# Autodesk Inventor assembly: Lower_wheel
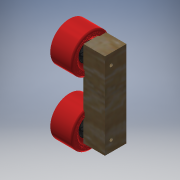
[picture p0: Inventor's stored thumbnail of the model, 180x180]
Saved by Autodesk Inventor 2016 SP2 (Build 200236200, 236)
## iProperties
Created: 2017-09-11
Part Number: Lower_wheel
Document SubType Name: Assembly
Designer: Admin
Author: Admin
## Documents named in this file (3)
- E:\DATA\Inventor\LinearMotion\Lower_wheel.iam
- E:\DATA\Inventor\LinearMotion\Blok_roda.ipt
- E:\DATA\Inventor\LinearMotion\90mm_wheel_asm.iam
## Components (3 placed, 2 different names)
1. Blok_roda:1 — Rotational:1, Rotational:2
2. 90mm_wheel_asm:1 [sub-assembly] — Rotational:1
3. 90mm_wheel_asm:2 [sub-assembly] — Rotational:2
## Relationships (2: RevoluteJoint 2)
- Rotational:1 [RevoluteJoint]: Blok_roda:1 ↔ 90mm_wheel_asm:1
- Rotational:2 [RevoluteJoint]: Blok_roda:1 ↔ 90mm_wheel_asm:2
